# Autodesk Inventor assembly: Upper_Leg_Left
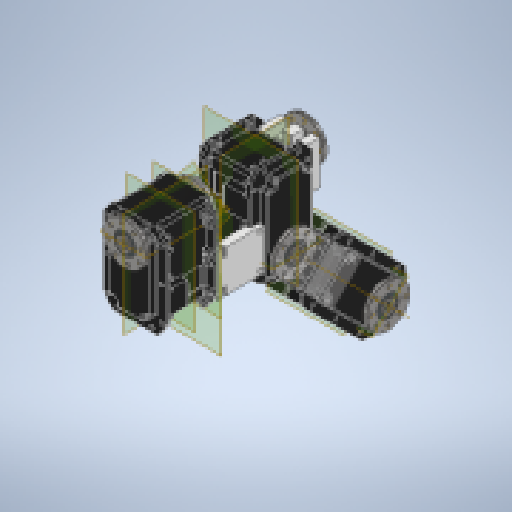
[picture p0: Inventor's stored thumbnail of the model, 512x512]
Saved by Autodesk Inventor 2024 (Build 280153000, 153)
## iProperties
Created: 2024-09-18
Part Number: Upper_Leg_Left
Document SubType Name: Assembly
Designer: Eungang
Author: Eungang
## Documents named in this file (8)
- C:\Users\Eungang\Documents\Inventor\FIGHTING_ROBOT_FINAL\부품\Upper_Leg_Left\Upper_Leg_Left.iam
- C:\Users\Eungang\Documents\Inventor\FIGHTING_ROBOT_FINAL\부품\Upper_Leg_Left\64-106_connect.ipt
- C:\Users\Eungang\Documents\Inventor\FIGHTING_ROBOT_FINAL\부품\아이들러\64아이들러.iam
- C:\Users\Eungang\Documents\Inventor\FIGHTING_ROBOT_FINAL\부품\혼\64-106Horn.ipt
- C:\Users\Eungang\Documents\Inventor\FIGHTING_ROBOT_FINAL\부품\Upper_Leg_Right\MX-106T.ipt
- C:\Users\Eungang\Documents\Inventor\FIGHTING_ROBOT_FINAL\부품\Upper_Leg_Right\knee_thighs_connect.ipt
- C:\Users\Eungang\Documents\Inventor\FIGHTING_ROBOT_FINAL\부품\Upper_Leg_Left\waist_thighs_bridge_MIR.ipt
- C:\Users\Eungang\Documents\Inventor\FIGHTING_ROBOT_FINAL\부품\다이나믹셀\MX-64T.ipt
## Components (15 placed, 7 different names)
1. 64-106_connect:1 — 삽입:18, 삽입:19, 삽입:24, 삽입:25
2. MX-106T:3
3. 64아이들러:3 [sub-assembly] — 삽입:27
4. 64-106Horn:3 — 삽입:26
5. 64아이들러:4 [sub-assembly]
6. 64-106Horn:4
7. MX-106T:4 — 삽입:15, 삽입:16, 삽입:18, 삽입:19, 삽입:20, 삽입:21
8. knee_thighs_connect:2 — 삽입:27, 각도:1
9. knee_thighs_connect:3 — 삽입:26
10. waist_thighs_bridge_MIR:1 — 삽입:15, 삽입:16, 삽입:17
11. 64아이들러:5 [sub-assembly] — 삽입:17
12. 64-106_connect:2 — 삽입:20, 삽입:21, 각도:1
13. MX-64T:1 — 삽입:24, 삽입:25
14. 64-106Horn:5
15. 64아이들러:6 [sub-assembly]
## Relationships (24: Insert 23, Angle 1)
- [Insert] (0.5 mm): MX-106T:3 ↔ 64-106Horn:4
- [Insert] (0.5 mm): MX-106T:3 ↔ 64아이들러:4
- [Insert] (0.5 mm): 64아이들러:3 ↔ MX-106T:4
- [Insert] (0.5 mm): 64-106Horn:3 ↔ MX-106T:4
- [Insert]: 64아이들러:3 ↔ knee_thighs_connect:2
- [Insert] (0.2 mm): MX-106T:3 ↔ knee_thighs_connect:2
- [Insert] (0.2 mm): MX-106T:3 ↔ knee_thighs_connect:2
- [Insert]: 64-106Horn:3 ↔ knee_thighs_connect:3
- [Insert] (0.2 mm): MX-106T:3 ↔ knee_thighs_connect:3
- [Insert] (0.2 mm): MX-106T:3 ↔ knee_thighs_connect:3
- 삽입:15 [Insert] (0.1 mm): MX-106T:4 ↔ waist_thighs_bridge_MIR:1
- 삽입:16 [Insert] (0.1 mm): MX-106T:4 ↔ waist_thighs_bridge_MIR:1
- 삽입:17 [Insert]: waist_thighs_bridge_MIR:1 ↔ 64아이들러:5
- 삽입:18 [Insert] (0.1 mm): 64-106_connect:1 ↔ MX-106T:4
- 삽입:19 [Insert] (0.1 mm): 64-106_connect:1 ↔ MX-106T:4
- 삽입:20 [Insert] (0.1 mm): MX-106T:4 ↔ 64-106_connect:2
- 삽입:21 [Insert] (0.1 mm): MX-106T:4 ↔ 64-106_connect:2
- [Insert] (0.5 mm): MX-64T:1 ↔ 64-106Horn:5
- [Insert] (0.5 mm): MX-64T:1 ↔ 64아이들러:6
- 삽입:24 [Insert] (0.1 mm): 64-106_connect:1 ↔ MX-64T:1
- 삽입:25 [Insert] (0.1 mm): 64-106_connect:1 ↔ MX-64T:1
- 삽입:26 [Insert]: 64-106Horn:3 ↔ knee_thighs_connect:3
- 삽입:27 [Insert]: 64아이들러:3 ↔ knee_thighs_connect:2
- 각도:1 [Angle] (315 deg): knee_thighs_connect:2 ↔ 64-106_connect:2
## Named parameters: d12_d1 = 0.5 mm
